# Autodesk Inventor assembly: base mg996r 3mm frame
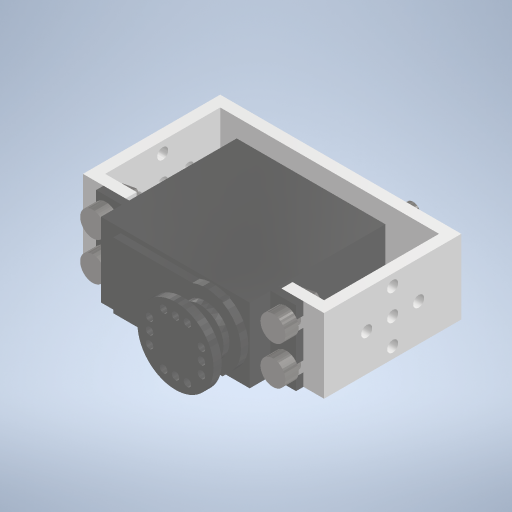
[picture p0: Inventor's stored thumbnail of the model, 512x512]
Saved by Autodesk Inventor 2023 (Build 270158000, 158)
## iProperties
Created: 2022-06-29
Part Number: base mg996r 3mm frame
Document SubType Name: Assembly
Designer: isamu
Author: isamu
## iProperties of the stored document Body003.ipt
Created: 2022-06-29
Part Number: Body003
Material: Generic
Document SubType Name: Modeling
Designer: isamu
Density: 1 g/cm^3
Appearance: Default
Author: isamu
## iProperties of the stored document servo frame.iam
Created: 2022-06-29
Part Number: servo frame
Description: FreeCAD Model
Document SubType Name: Assembly
Designer: isamu
Authority: Unknown
Sending System: FreeCAD
Preprocessor: Open CASCADE STEP processor 7.5
Title: Open CASCADE Shape Model
Author: Author
## Documents named in this file (9)
- D:\personal_projects\robot\inventor\base mg996r 3mm frame.iam
- D:\personal_projects\robot\exports\frames\servo-motor-mg966r.ipt
- **D:\personal_projects\robot\inventor\base mg996r 3mm frame.iam*LocalDocs*xAaaaavaaAaaaaaaaAaaaaiiwPc*servo frame.iam
- D:\personal_projects\robot\exports\frames\handle4.ipt
- D:\personal_projects\robot\exports\frames\m4x8.ipt
- D:\personal_projects\robot\exports\frames\m4 nuts.ipt
- D:\personal_projects\robot\exports\frames\m4x12.ipt
- **D:\personal_projects\robot\inventor\base mg996r 3mm frame.iam*LocalDocs*xAaaaadcaAaaaaaaaAaaaqe5xIh*Body003.ipt
- D:\personal_projects\robot\exports\frames\servo frame.step
## Components (13 placed, 6 different names)
1. servo-motor-mg966r:1 — Mate:1, Mate:2, Mate:3, Rotational:1, Insert:1, Insert:2, Insert:3, Insert:4
2. servo frame:1 [sub-assembly] — Mate:1, Mate:2, Mate:3, Insert:5, Insert:6, Insert:7, Insert:8, Insert:9, Insert:10
3. handle4:1 — Rotational:1
4. m4x8:1 — Insert:2
5. m4x8:2 — Insert:4
6. m4x8:3 — Insert:3
7. m4x8:4 — Insert:1
8. m4 nuts:1 — Insert:8
9. m4 nuts:2 — Insert:7
10. m4 nuts:3 — Insert:6
11. m4 nuts:4 — Insert:5
12. m4x12:1 — Insert:9
13. m4 nuts:5 — Insert:10
## Relationships (14: Insert 10, Mate 3, RevoluteJoint 1)
- Mate:1: servo-motor-mg966r:1 ↔ servo frame:1
- Mate:2: servo-motor-mg966r:1 ↔ servo frame:1
- Mate:3: servo-motor-mg966r:1 ↔ servo frame:1
- Rotational:1 [RevoluteJoint]: servo-motor-mg966r:1 ↔ handle4:1
- Insert:1: servo-motor-mg966r:1 ↔ m4x8:4
- Insert:2: servo-motor-mg966r:1 ↔ m4x8:1
- Insert:3: servo-motor-mg966r:1 ↔ m4x8:3
- Insert:4: servo-motor-mg966r:1 ↔ m4x8:2
- Insert:5: servo frame:1 ↔ m4 nuts:4
- Insert:6: servo frame:1 ↔ m4 nuts:3
- Insert:7: servo frame:1 ↔ m4 nuts:2
- Insert:8: servo frame:1 ↔ m4 nuts:1
- Insert:9: servo frame:1 ↔ m4x12:1
- Insert:10: servo frame:1 ↔ m4 nuts:5
